# Autodesk Inventor assembly: Bed Bracket 1.0
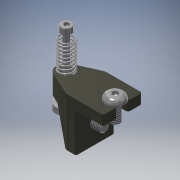
[picture p0: Inventor's stored thumbnail of the model, 180x180]
Saved by Autodesk Inventor 2016 (Build 200138000, 138)
## iProperties
Created: 2017-04-14
Part Number: Bed Bracket 1.0
Document SubType Name: Assembly
Designer: Scott
Author: Scott
## Documents named in this file (6)
- E:\Scott Projects\3D Printing\CoreXY\Bed Bracket 1.0.iam
- E:\Scott Projects\3D Printing\CoreXY\Mk2 Heat Bed Bracket.ipt
- E:\Scott Projects\3D Printing\CoreXY\Bed spring.ipt
- E:\Scott Projects\3D Printing\CoreXY\Bed Thumb Screw.ipt
- C:\Users\Scott\Documents\Inventor\Content Center Files\R2016\en-US\ANSI B18.3.1M(1)\ANSI B18.3.1M - M3x0.5 x 40(2).ipt
- C:\Users\Scott\Documents\Inventor\Content Center Files\R2016\en-US\ANSI B18.3.4M(1)\ANSI B18.3.4M - M5 x 0.8 x 10(2).ipt
## Components (6 placed, 5 different names)
1. Mk2 Heat Bed Bracket:1 — Mate:1, Flush:1, Insert:1, Insert:2, Insert:3, Insert:4
2. Bed spring:1 — Mate:1, Flush:1
3. Bed Thumb Screw:1 — Insert:1
4. Broached Socket Head Cap Screw - Metric M3x0.5 x 40:1 — Insert:2
5. Broached Hexagon Socket Button Head Cap Screw - Metric M5 x 0.8 x 10:1 — Insert:4
6. Broached Hexagon Socket Button Head Cap Screw - Metric M5 x 0.8 x 10:2 — Insert:3
## Relationships (6: Insert 4, Mate 1, Flush 1)
- Mate:1: Mk2 Heat Bed Bracket:1 ↔ Bed spring:1
- Flush:1: Mk2 Heat Bed Bracket:1 ↔ Bed spring:1
- Insert:1: Mk2 Heat Bed Bracket:1 ↔ Bed Thumb Screw:1
- Insert:2 (18 mm): Mk2 Heat Bed Bracket:1 ↔ Broached Socket Head Cap Screw - Metric M3x0.5 x 40:1
- Insert:3: Mk2 Heat Bed Bracket:1 ↔ Broached Hexagon Socket Button Head Cap Screw - Metric M5 x 0.8 x 10:2
- Insert:4: Mk2 Heat Bed Bracket:1 ↔ Broached Hexagon Socket Button Head Cap Screw - Metric M5 x 0.8 x 10:1
